# Autodesk Inventor assembly: Assembly1
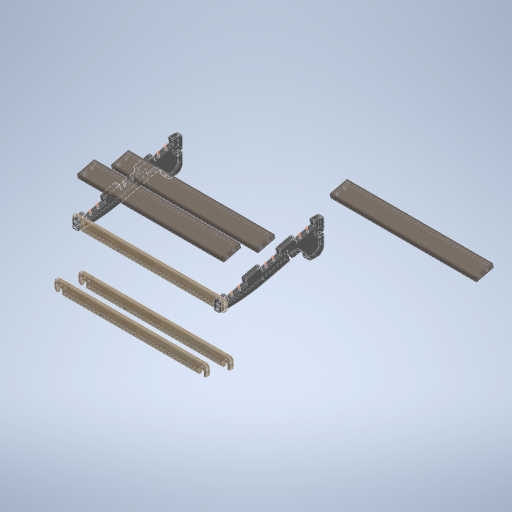
[picture p0: Inventor's stored thumbnail of the model, 512x512]
Saved by Autodesk Inventor 2023 (Build 270158030, 158C)
## iProperties
Created: 2022-12-16
Part Number: Assembly1
Document SubType Name: Assembly
Designer: Imogen Heard
Author: Imogen Heard
## Documents named in this file (6)
- C:\Users\dheard\Documents\Inventor\Inventor_Projects\Heriot Watt\CAD Porfolio\PedalBoard\Assembly1.iam
- C:\Users\dheard\Documents\Inventor\Inventor_Projects\Heriot Watt\CAD Porfolio\PedalBoard\Side.ipt
- C:\Users\dheard\Documents\Inventor\Inventor_Projects\Heriot Watt\CAD Porfolio\PedalBoard\Crossbar.ipt
- C:\Users\dheard\Documents\Inventor\Inventor_Projects\Heriot Watt\CAD Porfolio\PedalBoard\bracing.ipt
- C:\Users\dheard\Documents\Inventor\Inventor_Projects\Heriot Watt\CAD Porfolio\PedalBoard\Crossbar_CPY.ipt
- C:\Users\dheard\Documents\Inventor\Inventor_Projects\Heriot Watt\CAD Porfolio\PedalBoard\dowel.ipt
## Components (20 placed, 5 different names)
1. Side:1 — Mate:1, Mate:2, Mate:3, Mate:8, Insert:1, Insert:2, Insert:3, Insert:4, Insert:5, Insert:6
2. Crossbar:1
3. bracing:1 — Mate:1, Mate:2, Mate:3, Mate:4, Mate:5, Mate:6
4. Crossbar_CPY:1
5. Crossbar_CPY:2
6. bracing:2
7. bracing:3
8. dowel:1 — Mate:8, Insert:4
9. dowel:2 — Insert:9
10. dowel:3 — Insert:10
11. dowel:4 — Insert:2
12. dowel:5 — Insert:1
13. dowel:7 — Insert:5
14. dowel:8 — Insert:6
15. dowel:9 — Insert:11
16. dowel:10 — Insert:3
17. dowel:11 — Insert:12
18. Side:2 — Mate:4, Mate:5, Mate:6, Insert:7, Insert:8, Insert:9, Insert:10, Insert:11, Insert:12
19. dowel:12 — Insert:7
20. dowel:13 — Insert:8
## Relationships (19: Insert 12, Mate 7)
- Mate:1: Side:1 ↔ bracing:1
- Mate:2: Side:1 ↔ bracing:1
- Mate:3: Side:1 ↔ bracing:1
- Mate:4: bracing:1 ↔ Side:2
- Mate:5: bracing:1 ↔ Side:2
- Mate:6: bracing:1 ↔ Side:2
- Mate:8: Side:1 ↔ dowel:1
- Insert:1 (-7.5 mm): Side:1 ↔ dowel:5
- Insert:2 (-7.5 mm): Side:1 ↔ dowel:4
- Insert:3 (-7.5 mm): Side:1 ↔ dowel:10
- Insert:4 (-7.5 mm): Side:1 ↔ dowel:1
- Insert:5 (-7.5 mm): Side:1 ↔ dowel:7
- Insert:6 (-7.5 mm): Side:1 ↔ dowel:8
- Insert:7 (-7.5 mm): Side:2 ↔ dowel:12
- Insert:8 (-7.5 mm): Side:2 ↔ dowel:13
- Insert:9 (-7.5 mm): dowel:2 ↔ Side:2
- Insert:10 (-7.5 mm): dowel:3 ↔ Side:2
- Insert:11 (-7.5 mm): dowel:9 ↔ Side:2
- Insert:12 (-7.5 mm): dowel:11 ↔ Side:2
